# Autodesk Inventor assembly: doos
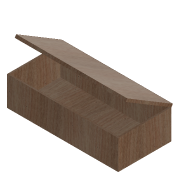
[picture p0: Inventor's stored thumbnail of the model, 180x180]
Saved by Autodesk Inventor 2020.3 (Build 243373000, 373)
## iProperties
Created: 2020-10-19
Part Number: doos
Document SubType Name: Assembly
Designer: Svend
Author: Svend
## Documents named in this file (5)
- C:\Users\Svend\OneDrive\Documents\GitHub\Rolstoel\doos.iam
- C:\Users\Svend\OneDrive\Documents\GitHub\Rolstoel\zijkant electronica.ipt
- C:\Users\Svend\OneDrive\Documents\GitHub\Rolstoel\zijkant2 electronica.ipt
- C:\Users\Svend\OneDrive\Documents\GitHub\Rolstoel\elektronica behuizing.ipt
- C:\Users\Svend\OneDrive\Documents\GitHub\Rolstoel\boevenkant doos.ipt
## Components (6 placed, 4 different names)
1. zijkant electronica:1 — Mate:5, Flush:3, Mate:6
2. zijkant2 electronica:1 — Mate:1, Mate:2, Flush:1
3. elektronica behuizing:1 — Mate:1, Mate:2, Flush:1, Mate:3, Mate:4, Flush:2, Mate:5, Flush:3, Mate:6, Mate:7, Flush:4, Mate:8
4. zijkant2 electronica:2 — Mate:3, Mate:4, Flush:2, Flush:7
5. zijkant electronica:2 — Mate:7, Flush:4, Mate:8, Mate:9
6. boevenkant doos:1 — Mate:9, Flush:7
## Relationships (14: Mate 9, Flush 5)
- Mate:1: zijkant2 electronica:1 ↔ elektronica behuizing:1
- Mate:2: zijkant2 electronica:1 ↔ elektronica behuizing:1
- Flush:1: zijkant2 electronica:1 ↔ elektronica behuizing:1
- Mate:3: elektronica behuizing:1 ↔ zijkant2 electronica:2
- Mate:4: elektronica behuizing:1 ↔ zijkant2 electronica:2
- Flush:2: elektronica behuizing:1 ↔ zijkant2 electronica:2
- Mate:5: zijkant electronica:1 ↔ elektronica behuizing:1
- Flush:3: zijkant electronica:1 ↔ elektronica behuizing:1
- Mate:6: zijkant electronica:1 ↔ elektronica behuizing:1
- Mate:7: elektronica behuizing:1 ↔ zijkant electronica:2
- Flush:4: elektronica behuizing:1 ↔ zijkant electronica:2
- Mate:8: elektronica behuizing:1 ↔ zijkant electronica:2
- Mate:9: zijkant electronica:2 ↔ boevenkant doos:1
- Flush:7: zijkant2 electronica:2 ↔ boevenkant doos:1
